# Autodesk Inventor assembly: Trabalho Final_999_001
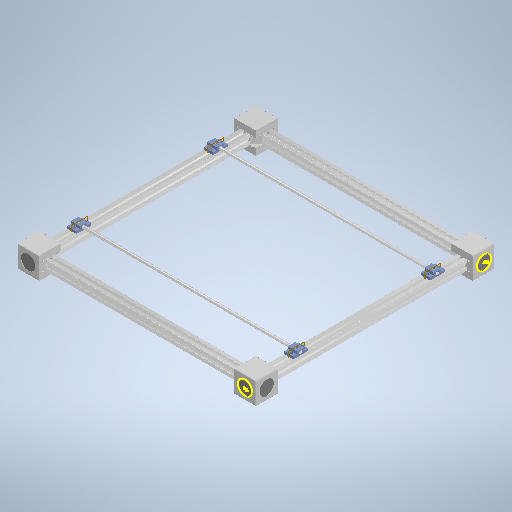
[picture p0: Inventor's stored thumbnail of the model, 512x512]
Saved by Autodesk Inventor 2026 (Build 300175000, 175)
## iProperties
Created: 2025-04-08
Part Number: Trabalho Final_999_001
Document SubType Name: Assembly
Designer: Carlos Dias
Author: Carlos Dias
## Documents named in this file (5)
- C:\Users\Tony Dias\Documents\Formação - IEFP\UFCDs\5134 - Robótica _ Fundamentos\Material De Apoio\Trabalho Final\Trabalho Final_999_001.iam
- C:\Users\Tony Dias\Documents\Formação - IEFP\UFCDs\5134 - Robótica _ Fundamentos\Material De Apoio\Trabalho Final\perfil_20x20_001.ipt
- C:\Users\Tony Dias\Documents\Formação - IEFP\UFCDs\5134 - Robótica _ Fundamentos\Material De Apoio\Trabalho Final\Design\CQC45452\CQC45452\CQC45452.ipt
- C:\Users\Tony Dias\Documents\Formação - IEFP\UFCDs\5134 - Robótica _ Fundamentos\Material De Apoio\Trabalho Final\suporte_veio_001_001.ipt
- C:\Users\Tony Dias\Documents\Formação - IEFP\UFCDs\5134 - Robótica _ Fundamentos\Material De Apoio\Trabalho Final\veio_001_001.ipt
## Components (14 placed, 4 different names)
1. perfil_20x20_001:1 — Mate:6, Mate:8, Mate:9, Angle:1, Mate:14, Mate:18, Mate:19, Mate:21, Mate:22
2. perfil_20x20_001:2 — Mate:10, Mate:15, Mate:16, Angle:5
3. perfil_20x20_001:3 — Mate:4, Mate:5, Mate:7, Mate:12, Angle:2, Angle:3
4. perfil_20x20_001:4 — Mate:1, Mate:2, Mate:11, Mate:13, Angle:4, Mate:23, Mate:24, Mate:26, Mate:28
5. CQC45452:1 — Mate:1, Mate:2, Mate:4, Mate:12, Flush:1, Mate:17, Flush:2, Angle:2, Angle:4
6. CQC45452:2 — Mate:5, Mate:6, Mate:7, Mate:8, Angle:3
7. CQC45452:4 — Mate:9, Mate:10, Angle:1, Mate:14, Mate:15, Mate:20
8. CQC45452:5 — Mate:11, Mate:13, Mate:16, Angle:5
9. suporte_veio_001_001:1 — Mate:18, Mate:19, Mate:20, Symmetry:1, Mate:25, Mate:31
10. suporte_veio_001_001:2 — Mate:21, Mate:22, Symmetry:1, Mate:27, Mate:30, Flush:3
11. suporte_veio_001_001:3 — Mate:23, Mate:24, Mate:25, Mate:32, Flush:4
12. suporte_veio_001_001:4 — Mate:26, Mate:27, Mate:28, Mate:29
13. veio_001_001:1 — Mate:29, Mate:30, Flush:3
14. veio_001_001:2 — Mate:31, Mate:32, Flush:4
## Relationships (41: Mate 31, Angle 5, Flush 4, Symmetry 1)
- Mate:1: perfil_20x20_001:4 ↔ CQC45452:1
- Mate:2: perfil_20x20_001:4 ↔ CQC45452:1
- Mate:4: perfil_20x20_001:3 ↔ CQC45452:1
- Mate:5: perfil_20x20_001:3 ↔ CQC45452:2
- Mate:6: perfil_20x20_001:1 ↔ CQC45452:2
- Mate:7: perfil_20x20_001:3 ↔ CQC45452:2
- Mate:8: perfil_20x20_001:1 ↔ CQC45452:2
- Mate:9: perfil_20x20_001:1 ↔ CQC45452:4
- Mate:10: perfil_20x20_001:2 ↔ CQC45452:4
- Mate:11: perfil_20x20_001:4 ↔ CQC45452:5
- Mate:12: perfil_20x20_001:3 ↔ CQC45452:1
- Mate:13: perfil_20x20_001:4 ↔ CQC45452:5
- Angle:1 (0 deg): perfil_20x20_001:1 ↔ CQC45452:4
- Mate:14: perfil_20x20_001:1 ↔ CQC45452:4
- Mate:15: perfil_20x20_001:2 ↔ CQC45452:4
- Mate:16: perfil_20x20_001:2 ↔ CQC45452:5
- Flush:1: CQC45452:1
- Mate:17: CQC45452:1
- Flush:2: CQC45452:1
- Angle:2 (0 deg): perfil_20x20_001:3 ↔ CQC45452:1
- Angle:3 (0 deg): perfil_20x20_001:3 ↔ CQC45452:2
- Angle:4 (0 deg): perfil_20x20_001:4 ↔ CQC45452:1
- Angle:5 (0 deg): perfil_20x20_001:2 ↔ CQC45452:5
- Mate:18: perfil_20x20_001:1 ↔ suporte_veio_001_001:1
- Mate:19: perfil_20x20_001:1 ↔ suporte_veio_001_001:1
- Mate:20 (45 mm): CQC45452:4 ↔ suporte_veio_001_001:1
- Mate:21: perfil_20x20_001:1 ↔ suporte_veio_001_001:2
- Mate:22: perfil_20x20_001:1 ↔ suporte_veio_001_001:2
- Symmetry:1: suporte_veio_001_001:1 ↔ suporte_veio_001_001:2
- Mate:23: perfil_20x20_001:4 ↔ suporte_veio_001_001:3
- Mate:24: perfil_20x20_001:4 ↔ suporte_veio_001_001:3
- Mate:25: suporte_veio_001_001:1 ↔ suporte_veio_001_001:3
- Mate:26: perfil_20x20_001:4 ↔ suporte_veio_001_001:4
- Mate:27: suporte_veio_001_001:2 ↔ suporte_veio_001_001:4
- Mate:28: perfil_20x20_001:4 ↔ suporte_veio_001_001:4
- Mate:29: suporte_veio_001_001:4 ↔ veio_001_001:1
- Mate:30: suporte_veio_001_001:2 ↔ veio_001_001:1
- Flush:3: suporte_veio_001_001:2 ↔ veio_001_001:1
- Mate:31: suporte_veio_001_001:1 ↔ veio_001_001:2
- Mate:32: suporte_veio_001_001:3 ↔ veio_001_001:2
- Flush:4: suporte_veio_001_001:3 ↔ veio_001_001:2
